# Autodesk Inventor assembly: YZ_GANTRY
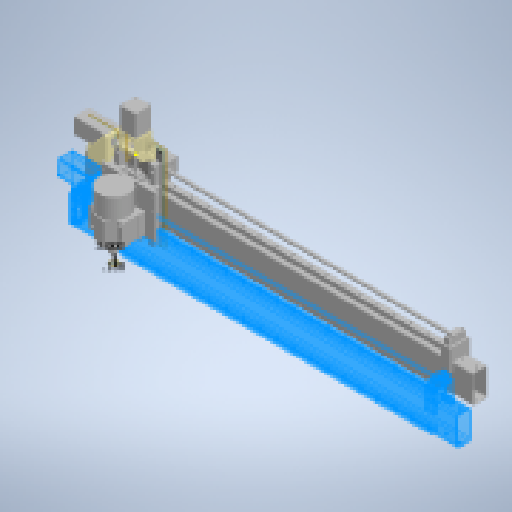
[picture p0: Inventor's stored thumbnail of the model, 512x512]
Saved by Autodesk Inventor 2023 (Build 270158000, 158)
## iProperties
Created: 2023-06-21
Part Number: YZ_GANTRY
Document SubType Name: Assembly
Designer: plebbb
Author: plebbb
## Documents named in this file (3)
- D:\Users\plebbb\Desktop\CNC_Project\YZ_GANTRY.iam
- D:\Users\plebbb\Desktop\CNC_Project\Z_GANTRY.iam
- D:\Users\plebbb\Desktop\CNC_Project\Y_GANTRY.iam
## Components (2 placed, 2 different names)
1. Z_GANTRY:1 [sub-assembly]
2. Y_GANTRY:1 [sub-assembly]
## Relationships (7: Mate 7)
- [Mate]: Z_GANTRY:1 ↔ Y_GANTRY:1
- [Mate]: Z_GANTRY:1 ↔ Y_GANTRY:1
- [Mate]: Z_GANTRY:1 ↔ Y_GANTRY:1
- [Mate]: Z_GANTRY:1 ↔ Y_GANTRY:1
- [Mate]: Z_GANTRY:1 ↔ Y_GANTRY:1
- [Mate]: Z_GANTRY:1 ↔ Y_GANTRY:1
- [Mate]: Z_GANTRY:1 ↔ Y_GANTRY:1
## Named parameters: d32_d65 = 0 mm, d33_d66 = 0 mm
